# Autodesk Inventor assembly: main_assembly
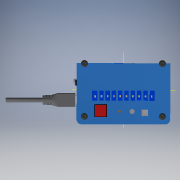
[picture p0: Inventor's stored thumbnail of the model, 180x180]
Saved by Autodesk Inventor 2016 (Build 200138000, 138)
## iProperties
Created: 2018-08-02
Part Number: main_assembly
Document SubType Name: Assembly
Designer: Luke
Author: Luke
## Documents named in this file (13)
- E:\CURRENT\PROJECTS\POMODORO\Mechanical\Assemblies\main_assembly.iam
- E:\CURRENT\PROJECTS\POMODORO\Mechanical\Parts\case_front.ipt
- E:\CURRENT\PROJECTS\POMODORO\Mechanical\Assemblies\Board\Board_Pomodoro_v1.0.iam
- E:\CURRENT\PROJECTS\POMODORO\Mechanical\Parts\Standard\Micro_usb_connector.ipt
- E:\CURRENT\PROJECTS\POMODORO\Mechanical\Parts\Standard\BATTERY_1S_560MAH_AKYGA.ipt
- E:\CURRENT\PROJECTS\POMODORO\Mechanical\Parts\case_back.ipt
- E:\CURRENT\PROJECTS\POMODORO\Mechanical\Parts\back_support.ipt
- E:\CURRENT\PROJECTS\POMODORO\Mechanical\Parts\Standard\knurled_insert_M2,5_4.ipt
- E:\CURRENT\PROJECTS\POMODORO\Mechanical\Parts\Standard\knurled_insert_M3_4.ipt
- C:\Users\Luke\Documents\Inventor\Content Center Files\R2016\en-US\ISO 7380-1\ISO 7380-1 - M3 x 16.ipt
- C:\Users\Luke\Documents\Inventor\Content Center Files\R2016\en-US\ISO 4762(2)\ISO 4762 - M2,5 x 8ISO.ipt
- E:\CURRENT\PROJECTS\POMODORO\Mechanical\Parts\Standard\Photoresistor\GL5528-Photoresistor.iam
- C:\Users\Luke\Documents\Inventor\Content Center Files\R2016\en-US\ISO 4035(2)\ISO 4035 - M3 - ISO.ipt
## Components (17 placed, 12 different names)
1. case_front:1 — Mate:5, Rotational:4, Rotational:5, Rotational:6, Rotational:7, Cylindrical:6, Cylindrical:7, Mate:8, Mate:12, Rotational:8
2. Board_Pomodoro_v1.0:1 [sub-assembly] — Cylindrical:6, Cylindrical:7, Mate:8, Mate:9, Mate:10, Mate:11, Cylindrical:8, Cylindrical:9
3. Micro_usb_connector:1 — Mate:9, Mate:10, Mate:11
4. BATTERY_1S_560MAH_AKYGA:1 — Mate:7
5. case_back:1 — Mate:5, Cylindrical:5, Mate:6, Rotational:1, Rotational:2, Rotational:3, Mate:7, Cylindrical:8, Rotational:9, Rotational:10
6. back_support:1 — Cylindrical:5, Mate:6
7. knurled_insert_M2,5_4:1 — Rotational:1
8. knurled_insert_M3_4:1 — Rotational:3
9. knurled_insert_M3_4:2 — Rotational:2, Cylindrical:9
10. ISO 7380-1 M3 x 16:1 — Rotational:5
11. ISO 7380-1 M3 x 16:2 — Rotational:4
12. ISO 7380-1 M3 x 16:3 — Rotational:8
13. ISO 7380-1 M3 x 16:4 — Rotational:6
14. ISO 4762 M2,5 x 8:1 — Rotational:7
15. GL5528-Photoresistor:1 [sub-assembly] — Mate:12
16. ISO 4035 M3:1 — Rotational:9
17. ISO 4035 M3:2 — Rotational:10
## Relationships (23: RevoluteJoint 10, Mate 8, CylindricalJoint 5)
- Mate:5: case_front:1 ↔ case_back:1
- Cylindrical:5: case_back:1 ↔ back_support:1
- Mate:6 (0.5 mm): case_back:1 ↔ back_support:1
- Rotational:1 [RevoluteJoint]: case_back:1 ↔ knurled_insert_M2,5_4:1
- Rotational:2 [RevoluteJoint]: case_back:1 ↔ knurled_insert_M3_4:2
- Rotational:3 [RevoluteJoint]: case_back:1 ↔ knurled_insert_M3_4:1
- Rotational:4 [RevoluteJoint]: case_front:1 ↔ ISO 7380-1 M3 x 16:2
- Rotational:5 [RevoluteJoint]: case_front:1 ↔ ISO 7380-1 M3 x 16:1
- Mate:7: BATTERY_1S_560MAH_AKYGA:1 ↔ case_back:1
- Rotational:6 [RevoluteJoint]: case_front:1 ↔ ISO 7380-1 M3 x 16:4
- Rotational:7 [RevoluteJoint]: case_front:1 ↔ ISO 4762 M2,5 x 8:1
- Cylindrical:6: case_front:1 ↔ Board_Pomodoro_v1.0:1
- Cylindrical:7: case_front:1 ↔ Board_Pomodoro_v1.0:1
- Mate:8: case_front:1 ↔ Board_Pomodoro_v1.0:1
- Mate:9: Board_Pomodoro_v1.0:1 ↔ Micro_usb_connector:1
- Mate:10: Board_Pomodoro_v1.0:1 ↔ Micro_usb_connector:1
- Mate:11: Board_Pomodoro_v1.0:1 ↔ Micro_usb_connector:1
- Cylindrical:8: Board_Pomodoro_v1.0:1 ↔ case_back:1
- Cylindrical:9: Board_Pomodoro_v1.0:1 ↔ knurled_insert_M3_4:2
- Mate:12: case_front:1 ↔ GL5528-Photoresistor:1
- Rotational:8 [RevoluteJoint]: case_front:1 ↔ ISO 7380-1 M3 x 16:3
- Rotational:9 [RevoluteJoint]: case_back:1 ↔ ISO 4035 M3:1
- Rotational:10 [RevoluteJoint]: case_back:1 ↔ ISO 4035 M3:2
